# Autodesk Inventor assembly: chaimber
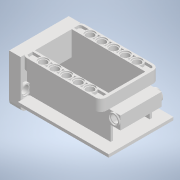
[picture p0: Inventor's stored thumbnail of the model, 180x180]
Saved by Autodesk Inventor 2021 (Build 250183000, 183)
## iProperties
Created: 2024-03-19
Part Number: chaimber
Document SubType Name: Assembly
Designer: 22hamfri
Author: 22hamfri
## Documents named in this file (4)
- C:\Users\22hamfri\Desktop\CAD\domino-1\chaimber.iam
- C:\Users\22hamfri\Desktop\CAD\domino-1\chaimber-adapter.ipt
- C:\Users\22hamfri\Desktop\CAD\domino-1\chaimber.ipt
- C:\Users\22hamfri\Desktop\CAD\domino-1\magazine-adapter.ipt
## Components (3 placed, 3 different names)
1. chaimber-adapter:1 — Rigid:1
2. chaimber:1 — Rigid:1, Rigid:3
3. magazine-adapter:1 — Rigid:3
## Relationships (2: WeldJoint 2)
- Rigid:1 [WeldJoint]: chaimber-adapter:1 ↔ chaimber:1
- Rigid:3 [WeldJoint]: chaimber:1 ↔ magazine-adapter:1
